# Autodesk Inventor assembly: Сборка129
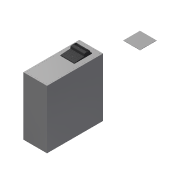
[picture p0: Inventor's stored thumbnail of the model, 180x180]
Saved by Autodesk Inventor 2017 (Build 210142000, 142)
## iProperties
Part Number: Сборка129
Material: Типовые
Document SubType Name: Assembly
Designer: Евтушенко
Author: Евтушенко
## Documents named in this file (9)
- D:\ИНИТ\Разработка\Терминалы\Express Pos Cash v.2\Сборка129.iam
- D:\ИНИТ\Разработка\Терминалы\Express Pos Cash v.2\00 - Прочее\MSM GX with Cassette 1500\MSM GX with Cassette 1500 and Bezel 78.ipt
- D:\ИНИТ\Разработка\Терминалы\Express Pos Cash v.2\Деталь135.ipt
- D:\ИНИТ\Разработка\Терминалы\Express Pos Cash v.2\Деталь136.ipt
- D:\ИНИТ\Разработка\Терминалы\Express Pos Cash v.2\Деталь137.ipt
- D:\ИНИТ\Разработка\Терминалы\Express Pos Cash v.2\Деталь138.ipt
- D:\ИНИТ\Разработка\Терминалы\Express Pos Cash v.2\Деталь139.ipt
- D:\ИНИТ\Разработка\Терминалы\Express Pos Cash v.2\Деталь140.ipt
- D:\ИНИТ\Разработка\Терминалы\Express Pos Cash v.2\Деталь141.ipt
## Components (8 placed, 8 different names)
1. MSM GX with Cassette 1500 and Bezel 78:1 — Совмещение:10
2. Деталь135:1 — Совмещение:1, Совмещение:2, Заподлицо:1, Заподлицо:3
3. Деталь136:1 — Совмещение:1, Заподлицо:1, Заподлицо:2, Заподлицо:3, Заподлицо:4, Заподлицо:5, Совмещение:3, Заподлицо:6, Совмещение:4, Заподлицо:7, Заподлицо:8, Совмещение:6
4. Деталь137:1 — Совмещение:2, Заподлицо:2, Заподлицо:4
5. Деталь138:1 — Заподлицо:5, Совмещение:3, Заподлицо:6, Совмещение:5, Заподлицо:10
6. Деталь139:1 — Совмещение:4, Заподлицо:7, Заподлицо:8
7. Деталь140:1 — Совмещение:5, Совмещение:6, Заподлицо:10, Совмещение:10
8. Деталь141:1
## Relationships (16: Flush 9, Mate 7)
- Совмещение:1 [Mate] (1 mm): Деталь135:1 ↔ Деталь136:1
- Совмещение:2 [Mate] (1 mm): Деталь135:1 ↔ Деталь137:1
- Заподлицо:1 [Flush] (-1 mm): Деталь135:1 ↔ Деталь136:1
- Заподлицо:2 [Flush]: Деталь136:1 ↔ Деталь137:1
- Заподлицо:3 [Flush]: Деталь135:1 ↔ Деталь136:1
- Заподлицо:4 [Flush]: Деталь136:1 ↔ Деталь137:1
- Заподлицо:5 [Flush]: Деталь136:1 ↔ Деталь138:1
- Совмещение:3 [Mate]: Деталь136:1 ↔ Деталь138:1
- Заподлицо:6 [Flush]: Деталь136:1 ↔ Деталь138:1
- Совмещение:4 [Mate]: Деталь136:1 ↔ Деталь139:1
- Заподлицо:7 [Flush]: Деталь136:1 ↔ Деталь139:1
- Заподлицо:8 [Flush]: Деталь136:1 ↔ Деталь139:1
- Совмещение:10 [Mate]: MSM GX with Cassette 1500 and Bezel 78:1 ↔ Деталь140:1
- Совмещение:5 [Mate]: Деталь138:1 ↔ Деталь140:1
- Совмещение:6 [Mate]: Деталь136:1 ↔ Деталь140:1
- Заподлицо:10 [Flush]: Деталь138:1 ↔ Деталь140:1
